# Autodesk Inventor assembly: FirstAssembly
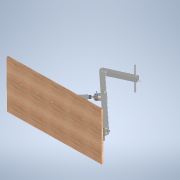
[picture p0: Inventor's stored thumbnail of the model, 180x180]
Saved by Autodesk Inventor 2022 (Build 260153000, 153)
## iProperties
Created: 2022-04-08
Part Number: FirstAssembly
Document SubType Name: Assembly
Designer: Patrick
Author: Patrick
## Documents named in this file (25)
- C:\Users\patri\OneDrive - Syddansk Universitet\2. Semester Master\Mekaniske Elementer\Mini Project\2020-10-23\Workspaces\Workspace\FirstAssembly.iam
- C:\Users\patri\OneDrive - Syddansk Universitet\2. Semester Master\Mekaniske Elementer\Mini Project\2020-10-23\Workspaces\Workspace\IMS-10-001.ipt
- C:\Users\patri\OneDrive - Syddansk Universitet\2. Semester Master\Mekaniske Elementer\Mini Project\2020-10-23\Workspaces\Workspace\IMS-00-003.ipt
- C:\Users\patri\OneDrive - Syddansk Universitet\2. Semester Master\Mekaniske Elementer\Mini Project\2020-10-23\Workspaces\Workspace\IMS-10-002.ipt
- C:\Users\patri\OneDrive - Syddansk Universitet\2. Semester Master\Mekaniske Elementer\Mini Project\2020-10-23\Workspaces\Workspace\Bund_beslag\Beslag_til_stempel'.iam
- C:\Users\patri\OneDrive - Syddansk Universitet\2. Semester Master\Mekaniske Elementer\Mini Project\2020-10-23\Workspaces\Workspace\Beam\Beam_v3.iam
- C:\Users\patri\OneDrive - Syddansk Universitet\2. Semester Master\Mekaniske Elementer\Mini Project\2020-10-23\Workspaces\Workspace\Bushings\Bøsning_beam_bund.ipt
- C:\Users\patri\OneDrive - Syddansk Universitet\2. Semester Master\Mekaniske Elementer\Mini Project\2020-10-23\Workspaces\Workspace\Aksler\potentiometer_aksel.ipt
- C:\Users\patri\OneDrive - Syddansk Universitet\2. Semester Master\Mekaniske Elementer\Mini Project\2020-10-23\Libraries\Content Center Files\en-US\DIN 6921\DIN 6921 - M8 x 35 - B.ipt
- C:\Users\patri\OneDrive - Syddansk Universitet\2. Semester Master\Mekaniske Elementer\Mini Project\2020-10-23\Workspaces\Workspace\Beslag_potentiometer.ipt
- C:\Users\patri\OneDrive - Syddansk Universitet\2. Semester Master\Mekaniske Elementer\Mini Project\2020-10-23\Workspaces\Workspace\Beslag_beam_cylinder\Beam_stempel_beslag.iam
- C:\Users\patri\OneDrive - Syddansk Universitet\2. Semester Master\Mekaniske Elementer\Mini Project\2020-10-23\Workspaces\Workspace\Extra_Beam\Exstra håndtag.iam
- C:\Users\patri\OneDrive - Syddansk Universitet\2. Semester Master\Mekaniske Elementer\Mini Project\2020-10-23\Workspaces\Workspace\Håndtag.ipt
- C:\Users\patri\OneDrive - Syddansk Universitet\2. Semester Master\Mekaniske Elementer\Mini Project\2020-10-23\Workspaces\Workspace\Pin.ipt
- C:\Users\patri\OneDrive - Syddansk Universitet\2. Semester Master\Mekaniske Elementer\Mini Project\2020-10-23\Workspaces\Workspace\Stempel\193993 DSNU-40-300-P---(A---00--0-KS).ipt
- C:\Users\patri\OneDrive - Syddansk Universitet\2. Semester Master\Mekaniske Elementer\Mini Project\2020-10-23\Workspaces\Workspace\Stempel\193993 DSNU-40-300-P---(A----0-ZR).ipt
- C:\Users\patri\OneDrive - Syddansk Universitet\2. Semester Master\Mekaniske Elementer\Mini Project\2020-10-23\Workspaces\Workspace\Stempel\DIN-439-B - M12x1_25(F).ipt
- C:\Users\patri\OneDrive - Syddansk Universitet\2. Semester Master\Mekaniske Elementer\Mini Project\2020-10-23\Workspaces\Workspace\Stempel\IMS-01-001.ipt
- C:\Users\patri\OneDrive - Syddansk Universitet\2. Semester Master\Mekaniske Elementer\Mini Project\2020-10-23\Workspaces\Workspace\Bushings\Ydre_bøsning_stempel_stang.ipt
- C:\Users\patri\OneDrive - Syddansk Universitet\2. Semester Master\Mekaniske Elementer\Mini Project\2020-10-23\Workspaces\Workspace\Bushings\Indre_bøsning_Stempel_stang.ipt
- C:\Users\patri\OneDrive - Syddansk Universitet\2. Semester Master\Mekaniske Elementer\Mini Project\2020-10-23\Workspaces\Workspace\10mmPins.ipt
- C:\Users\patri\OneDrive - Syddansk Universitet\2. Semester Master\Mekaniske Elementer\Mini Project\2020-10-23\Workspaces\Workspace\Håndtag_til_pins.ipt
- C:\Users\patri\OneDrive - Syddansk Universitet\2. Semester Master\Mekaniske Elementer\Mini Project\2020-10-23\Libraries\Content Center Files\en-US\AS 1110\AS 1110 - M3 x 6.ipt
- C:\Users\patri\OneDrive - Syddansk Universitet\2. Semester Master\Mekaniske Elementer\Mini Project\2020-10-23\Workspaces\Workspace\Aksel_stempel_bund.ipt
- C:\Users\patri\OneDrive - Syddansk Universitet\2. Semester Master\Mekaniske Elementer\Mini Project\2020-10-23\Workspaces\Workspace\Bushings\Bushing_stempel.ipt
## Components (29 placed, 24 different names)
1. Beam_v3:1 [sub-assembly] — Cylindrical:3, Mate:5, Rotational:3, Rigid:5, Rotational:4
2. potentiometer_aksel:1 — Cylindrical:4, Mate:5
3. DIN 6921 M8 x 35:1 — Rotational:3
4. Beslag_potentiometer:1 — Mate:6, Flush:3, Flush:4
5. Beam_stempel_beslag:1 [sub-assembly] — Rigid:5, Cylindrical:7, Rotational:6, Rotational:7, Rotational:14
6. Exstra håndtag:1 [sub-assembly] — Rotational:4, Rotational:5
7. Håndtag:1 — Rotational:5, Mate:7, Mate:8
8. Pin til håndtag — Mate:7, Mate:8
9. 10mmPins:1 — Rotational:10
10. Håndtag_til_pins:1 — Rigid:6, Rotational:14
11. AS 1110 - Metric M3 x 6:1 — Rigid:6
12. Aksel_stempel_bund:1 — Rotational:13
13. Bushing_stempel:1 — Rotational:12, Rotational:13
14. Bushing_stempel:2 — Rotational:11
15. ClampOnBoard — Rigid:2, Rigid:4
16. BaseBoard — Rigid:2
17. ThreadsBaseBoard — Rigid:4, Mate:1, Flush:1, Flush:2, Mate:2, Mate:3, Mate:4, Flush:4
18. Beslag_til_stempel':1 [sub-assembly] — Mate:1, Flush:1, Flush:2, Cylindrical:3, Rotational:1, Rotational:2, Mate:6, Flush:3
19. Beslag_til_stempel':2 [sub-assembly] — Mate:2, Mate:3, Mate:4, Cylindrical:6, Rotational:11, Rotational:12
20. Bøsning_beam_bund:1 — Rotational:1
21. Bøsning_beam_bund:2 — Rotational:2, Cylindrical:4
22. 193993 DSNU-40-300-P---(A---00--0-KS):1 — Cylindrical:5, Mate:9, Mate:10, Mate:11
23. 193993 DSNU-40-300-P---(A----0-ZR):1 — Cylindrical:5, Cylindrical:6
24. DIN-439-B - M12x1_25(F):1 — Mate:9, Mate:10, Mate:12
25. IMS-01-001:1 — Mate:11, Mate:12, Cylindrical:7, Rotational:8, Rotational:9
26. Ydre_bøsning_stempel_stang:1 — Rotational:6
27. Ydre_bøsning_stempel_stang:2 — Rotational:7, Rotational:10
28. Indre_bøsning_Stempel_stang:1 — Rotational:9
29. Indre_bøsning_Stempel_stang:2 — Rotational:8
## Relationships (39: RevoluteJoint 14, Mate 12, CylindricalJoint 5, WeldJoint 4, Flush 4)
- Rigid:2 [WeldJoint]: ClampOnBoard ↔ BaseBoard
- Rigid:4 [WeldJoint]: ClampOnBoard ↔ ThreadsBaseBoard
- Mate:1: ThreadsBaseBoard ↔ Beslag_til_stempel':1
- Flush:1: ThreadsBaseBoard ↔ Beslag_til_stempel':1
- Flush:2: ThreadsBaseBoard ↔ Beslag_til_stempel':1
- Mate:2: ThreadsBaseBoard ↔ Beslag_til_stempel':2
- Mate:3: ThreadsBaseBoard ↔ Beslag_til_stempel':2
- Mate:4: ThreadsBaseBoard ↔ Beslag_til_stempel':2
- Cylindrical:3: Beam_v3:1 ↔ Beslag_til_stempel':1
- Rotational:1 [RevoluteJoint]: Beslag_til_stempel':1 ↔ Bøsning_beam_bund:1
- Rotational:2 [RevoluteJoint]: Beslag_til_stempel':1 ↔ Bøsning_beam_bund:2
- Cylindrical:4: potentiometer_aksel:1 ↔ Bøsning_beam_bund:2
- Mate:5: Beam_v3:1 ↔ potentiometer_aksel:1
- Rotational:3 [RevoluteJoint]: Beam_v3:1 ↔ DIN 6921 M8 x 35:1
- Mate:6: Beslag_potentiometer:1 ↔ Beslag_til_stempel':1
- Flush:3: Beslag_potentiometer:1 ↔ Beslag_til_stempel':1
- Flush:4 (2.5 mm): Beslag_potentiometer:1 ↔ ThreadsBaseBoard
- Rigid:5 [WeldJoint]: Beam_v3:1 ↔ Beam_stempel_beslag:1
- Rotational:4 [RevoluteJoint]: Beam_v3:1 ↔ Exstra håndtag:1
- Rotational:5 [RevoluteJoint]: Exstra håndtag:1 ↔ Håndtag:1
- Mate:7: Håndtag:1 ↔ Pin til håndtag
- Mate:8: Håndtag:1 ↔ Pin til håndtag
- Cylindrical:5: 193993 DSNU-40-300-P---(A---00--0-KS):1 ↔ 193993 DSNU-40-300-P---(A----0-ZR):1
- Mate:9: 193993 DSNU-40-300-P---(A---00--0-KS):1 ↔ DIN-439-B - M12x1_25(F):1
- Mate:10 (4 mm): 193993 DSNU-40-300-P---(A---00--0-KS):1 ↔ DIN-439-B - M12x1_25(F):1
- Mate:11: 193993 DSNU-40-300-P---(A---00--0-KS):1 ↔ IMS-01-001:1
- Mate:12: DIN-439-B - M12x1_25(F):1 ↔ IMS-01-001:1
- Cylindrical:6: Beslag_til_stempel':2 ↔ 193993 DSNU-40-300-P---(A----0-ZR):1
- Cylindrical:7: Beam_stempel_beslag:1 ↔ IMS-01-001:1
- Rotational:6 [RevoluteJoint]: Beam_stempel_beslag:1 ↔ Ydre_bøsning_stempel_stang:1
- Rotational:7 [RevoluteJoint]: Beam_stempel_beslag:1 ↔ Ydre_bøsning_stempel_stang:2
- Rotational:8 [RevoluteJoint]: IMS-01-001:1 ↔ Indre_bøsning_Stempel_stang:2
- Rotational:9 [RevoluteJoint]: IMS-01-001:1 ↔ Indre_bøsning_Stempel_stang:1
- Rotational:10 [RevoluteJoint]: 10mmPins:1 ↔ Ydre_bøsning_stempel_stang:2
- Rigid:6 [WeldJoint]: Håndtag_til_pins:1 ↔ AS 1110 - Metric M3 x 6:1
- Rotational:11 [RevoluteJoint]: Bushing_stempel:2 ↔ Beslag_til_stempel':2
- Rotational:12 [RevoluteJoint]: Bushing_stempel:1 ↔ Beslag_til_stempel':2
- Rotational:13 [RevoluteJoint] (-1 mm): Aksel_stempel_bund:1 ↔ Bushing_stempel:1
- Rotational:14 [RevoluteJoint]: Beam_stempel_beslag:1 ↔ Håndtag_til_pins:1
